# Autodesk Inventor assembly: joint
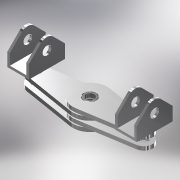
[picture p0: Inventor's stored thumbnail of the model, 180x180]
Saved by Autodesk Inventor 2018.2 (Build 222227000, 227)
## iProperties
Created: 2017-12-11
Part Number: joint
Material: 一般
Document SubType Name: Assembly
Designer: kuwano
Mass: 80.9259 g
Surface Area: 250.334 cm^2
Volume: 30.4872 cm^3
Density: 2.65442 g/cm^3
Author: kuwano
## Documents named in this file (4)
- D:\kuwano\Documents\Inventor\KITformula\AeroCAD2018\CAD\Inventor\製作用CAD\R-wing\parts\joint\joint.iam
- D:\kuwano\Documents\Inventor\KITformula\AeroCAD2018\CAD\Inventor\製作用CAD\R-wing\parts\joint\parts\plate.ipt
- D:\kuwano\Documents\Inventor\KITformula\AeroCAD2018\CAD\Inventor\製作用CAD\R-wing\parts\joint\parts\MF128ZZ.ipt
- D:\kuwano\Documents\Inventor\KITformula\AeroCAD2018\CAD\Inventor\製作用CAD\R-wing\parts\joint\parts\clip.ipt
## Components (10 placed, 3 different names)
1. plate:1 — メイト:5, メイト:7, メイト:8, メイト:11, メイト:12, メイト:15, フラッシュ:3, メイト:22
2. plate:2 — メイト:6, メイト:8, メイト:9, メイト:10, メイト:11, メイト:16, フラッシュ:4, メイト:18, メイト:21, メイト:22
3. plate:3 — メイト:5, メイト:9, メイト:10, メイト:13, メイト:17, フラッシュ:5, メイト:19, メイト:20
4. plate:4 — フラッシュ:1, メイト:6, メイト:7, メイト:12, メイト:14, フラッシュ:2
5. MF128ZZ:1 — メイト:17, フラッシュ:5
6. MF128ZZ:2 — メイト:16, フラッシュ:4
7. MF128ZZ:3 — メイト:15, フラッシュ:3
8. MF128ZZ:4 — メイト:14, フラッシュ:2
9. clip:1 — メイト:19, メイト:20, 角度:1, フラッシュ:6
10. clip:2 — メイト:18, メイト:21, 角度:1, フラッシュ:6
## Relationships (25: Mate 18, Flush 6, Angle 1)
- フラッシュ:1 [Flush]: plate:4
- メイト:5 [Mate]: plate:1 ↔ plate:3
- メイト:6 [Mate]: plate:2 ↔ plate:4
- メイト:7 [Mate] (1 mm): plate:1 ↔ plate:4
- メイト:8 [Mate] (1 mm): plate:1 ↔ plate:2
- メイト:9 [Mate] (1 mm): plate:2 ↔ plate:3
- メイト:10 [Mate]: plate:2 ↔ plate:3
- メイト:11 [Mate]: plate:1 ↔ plate:2
- メイト:12 [Mate]: plate:1 ↔ plate:4
- メイト:13 [Mate]: plate:3
- メイト:14 [Mate]: plate:4 ↔ MF128ZZ:4
- フラッシュ:2 [Flush]: plate:4 ↔ MF128ZZ:4
- メイト:15 [Mate]: plate:1 ↔ MF128ZZ:3
- フラッシュ:3 [Flush]: plate:1 ↔ MF128ZZ:3
- メイト:16 [Mate]: plate:2 ↔ MF128ZZ:2
- フラッシュ:4 [Flush]: plate:2 ↔ MF128ZZ:2
- メイト:17 [Mate]: plate:3 ↔ MF128ZZ:1
- フラッシュ:5 [Flush]: plate:3 ↔ MF128ZZ:1
- メイト:18 [Mate]: plate:2 ↔ clip:2
- メイト:19 [Mate]: plate:3 ↔ clip:1
- メイト:20 [Mate] (2 mm): plate:3 ↔ clip:1
- メイト:21 [Mate] (6.5 mm): plate:2 ↔ clip:2
- 角度:1 [Angle] (0 deg): clip:1 ↔ clip:2
- フラッシュ:6 [Flush]: clip:1 ↔ clip:2
- メイト:22 [Mate]: plate:1 ↔ plate:2
